# Autodesk Inventor assembly: Ensamble bomba
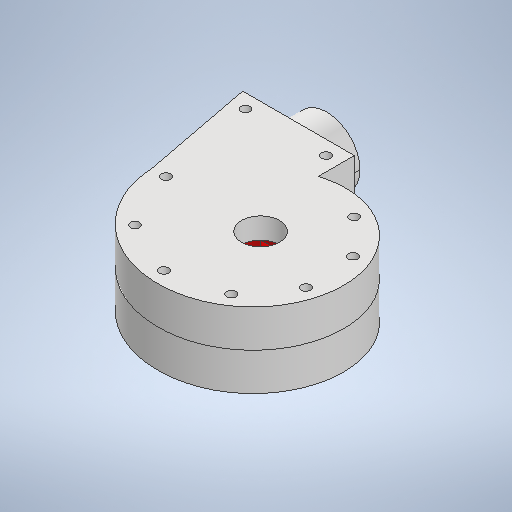
[picture p0: Inventor's stored thumbnail of the model, 512x512]
Saved by Autodesk Inventor 2025.3 (Build 293356000, 356)
## iProperties
Created: 2025-11-12
Part Number: Ensamble bomba
Document SubType Name: Assembly
Designer: juanm
Author: juanm
## Documents named in this file (4)
- C:\Users\juanm\Documents\Inventor\Turbo\Ensamble bomba.iam
- C:\Users\juanm\Documents\Inventor\Turbo\Rodete_4000RPM_2LS.ipt
- C:\Users\juanm\Documents\Inventor\Turbo\Base voluta.ipt
- C:\Users\juanm\Documents\Inventor\Turbo\Tapa voluta.ipt
## Components (3 placed, 3 different names)
1. Rodete_4000RPM_2LS:1 — Insert:1
2. Base voluta:1 — Insert:1, Flush:1, Mate:1, Flush:2
3. Tapa voluta:1 — Flush:1, Mate:1, Flush:2
## Relationships (4: Flush 2, Insert 1, Mate 1)
- Insert:1 (0.5 mm): Rodete_4000RPM_2LS:1 ↔ Base voluta:1
- Flush:1: Base voluta:1 ↔ Tapa voluta:1
- Mate:1: Base voluta:1 ↔ Tapa voluta:1
- Flush:2: Base voluta:1 ↔ Tapa voluta:1
